# Autodesk Inventor assembly: Test_assembly
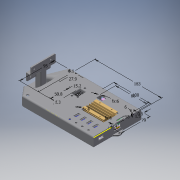
[picture p0: Inventor's stored thumbnail of the model, 180x180]
Saved by Autodesk Inventor 2019 (Build 230136000, 136)
## iProperties
Created: 2020-02-14
Part Number: Test_assembly
Document SubType Name: Assembly
Designer: close
Author: close
## Documents named in this file (8)
- C:\Users\close\Desktop\CAD BARC-ROAR\barc_hardware\Enclosure\V_4\Test_assembly_v4.iam
- C:\Users\close\Desktop\CAD BARC-ROAR\barc_hardware\Enclosure\V_4\Enclosure_v4.ipt
- C:\Users\close\Desktop\CAD BARC-ROAR\barc_hardware\Dependencies\Nvidia Jetson Nano\P3450_P3449_A02_P3448_A02.iam
- C:\Users\close\Desktop\CAD BARC-ROAR\barc_hardware\Dependencies\Splitter Board\SplitterBoard.iam
- C:\Users\close\Desktop\CAD BARC-ROAR\barc_hardware\Dependencies\Arduino\Mega\arduinoMegaDetailed.ipt
- C:\Users\close\Desktop\CAD BARC-ROAR\barc_hardware\Dependencies\Drok Step Down\CN2596-2.iam
- C:\Users\close\Desktop\CAD BARC-ROAR\barc_hardware\Enclosure\V_4\Camera Mount 30mm.ipt
- C:\Users\close\Desktop\CAD BARC-ROAR\barc_hardware\Enclosure\V_4\Dual Camera Mount.ipt
## Components (7 placed, 7 different names)
1. Enclosure_v4:1 — Insert:1, Insert:2, Insert:3, Insert:4, Insert:5, Insert:7, Insert:8, Insert:10, Flush:1
2. P3450_P3449_A02_P3448_A02:1 [sub-assembly] — Insert:1, Insert:2
3. SplitterBoard:1 [sub-assembly] — Insert:3, Insert:4
4. arduinoMegaDetailed:1 — Insert:5
5. CN2596-2:1 [sub-assembly] — Insert:7, Insert:8
6. Camera Mount 30mm:1 — Insert:10, Flush:1, Insert:11, Flush:2
7. Dual Camera Mount:1 — Insert:11, Flush:2
## Relationships (11: Insert 9, Flush 2)
- Insert:1: Enclosure_v4:1 ↔ P3450_P3449_A02_P3448_A02:1
- Insert:2: Enclosure_v4:1 ↔ P3450_P3449_A02_P3448_A02:1
- Insert:3: Enclosure_v4:1 ↔ SplitterBoard:1
- Insert:4: Enclosure_v4:1 ↔ SplitterBoard:1
- Insert:5: Enclosure_v4:1 ↔ arduinoMegaDetailed:1
- Insert:7: Enclosure_v4:1 ↔ CN2596-2:1
- Insert:8: Enclosure_v4:1 ↔ CN2596-2:1
- Insert:10: Enclosure_v4:1 ↔ Camera Mount 30mm:1
- Flush:1 (17 mm): Enclosure_v4:1 ↔ Camera Mount 30mm:1
- Insert:11: Camera Mount 30mm:1 ↔ Dual Camera Mount:1
- Flush:2: Camera Mount 30mm:1 ↔ Dual Camera Mount:1
